# Autodesk Inventor assembly: printer power brick assembly
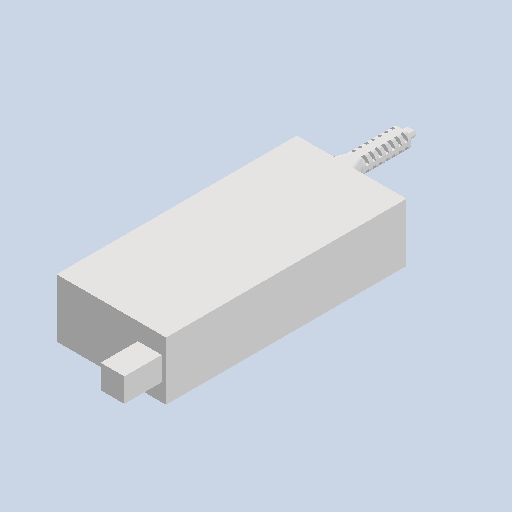
[picture p0: Inventor's stored thumbnail of the model, 512x512]
Saved by Autodesk Inventor 2022 (Build 260153000, 153)
## iProperties
Created: 2021-12-03
Part Number: printer power brick assembly
Document SubType Name: Assembly
Designer: efred
Author: efred
## Documents named in this file (3)
- C:\Users\efred\OneDrive - Imperial College London\ROBOICP\Linear Rail Assembly\printer power brick assembly.iam
- C:\Users\efred\OneDrive - Imperial College London\ROBOICP\Linear Rail Assembly\IEC C7 2P 2,5A 250V 4 180°.ipt
- C:\Users\efred\OneDrive - Imperial College London\ROBOICP\Linear Rail Assembly\Printer power brick.ipt
## Components (2 placed, 2 different names)
1. IEC C7 2P 2,5A 250V 4 180°:1 — Mate:1, Flush:1, Mate:3
2. Printer power brick:1 — Mate:1, Flush:1, Mate:3
## Relationships (3: Mate 2, Flush 1)
- Mate:1: IEC C7 2P 2,5A 250V 4 180°:1 ↔ Printer power brick:1
- Flush:1 (10 mm): IEC C7 2P 2,5A 250V 4 180°:1 ↔ Printer power brick:1
- Mate:3 (-15 mm): IEC C7 2P 2,5A 250V 4 180°:1 ↔ Printer power brick:1
